# Autodesk Inventor assembly: PolarizationMethod
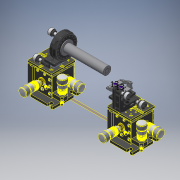
[picture p0: Inventor's stored thumbnail of the model, 180x180]
Saved by Autodesk Inventor 2019 (Build 230136000, 136)
## iProperties
Created: 2019-05-24
Part Number: PolarizationMethod
Document SubType Name: Assembly
Designer: aorfi
Author: aorfi
## Documents named in this file (10)
- C:\Users\aorfi\Documents\IQC\PolarizationMethod.iam
- C:\Users\aorfi\Documents\IQC\COTS\ThorLabs\3AxisStage-MBT616D.ipt
- C:\Users\aorfi\Documents\IQC\COTS\ThorLabs\RollStage-RSP1_M.ipt
- C:\Users\aorfi\Documents\IQC\COTS\ThorLabs\YawPitchStage-KM100PM.ipt
- C:\Users\aorfi\Documents\IQC\ChipMountAssembly.iam
- C:\Users\aorfi\Documents\IQC\COTS\Newport\LinearStage-MS-125-X.ipt
- C:\Users\aorfi\Documents\IQC\CustomParts\FiberMount.ipt
- C:\Users\aorfi\Documents\IQC\CustomParts\EpoxyFiberMountBase.ipt
- C:\Users\aorfi\Documents\IQC\CustomParts\FixedFiber.ipt
- C:\Users\aorfi\Documents\IQC\CustomParts\RubayetChip.ipt
## Components (12 placed, 9 different names)
1. 3AxisStage-MBT616D:1 — Mate:1, Flush:1, Mate:2, Flush:3, Flush:5
2. 3AxisStage-MBT616D:2 — Mate:6, Flush:4, Flush:5, Mate:8, Mate:12, Flush:7
3. RollStage-RSP1_M:1 — Mate:4, Angle:1, Mate:5, Mate:7, Mate:13, Mate:14
4. YawPitchStage-KM100PM:1 — Mate:2, Mate:4, Angle:1, Mate:13
5. ChipMountAssembly:1 [sub-assembly] — Mate:5, Mate:7
6. YawPitchStage-KM100PM:2 — Mate:8, Mate:10, Mate:12, Flush:6, Flush:7
7. LinearStage-MS-125-X:1 — Mate:10, Mate:11, Flush:6, Mate:16, Mate:17, Mate:18, Mate:19, Mate:20, Mate:21
8. FiberMount:1 — Mate:16, Flush:9, Mate:24, Mate:25, Mate:26, Flush:10
9. EpoxyFiberMountBase:1 — Mate:17, Mate:18, Mate:19, Flush:9, Mate:24
10. FixedFiber:1 — Mate:20, Mate:21, Mate:22, Mate:23, Flush:8
11. RubayetChip:1 — Mate:22, Mate:23, Flush:8
12. RubayetChip:2 — Mate:25, Mate:26, Flush:10
## Relationships (33: Mate 23, Flush 9, Angle 1)
- Mate:1: 3AxisStage-MBT616D:1
- Flush:1: 3AxisStage-MBT616D:1
- Mate:2: 3AxisStage-MBT616D:1 ↔ YawPitchStage-KM100PM:1
- Mate:4: RollStage-RSP1_M:1 ↔ YawPitchStage-KM100PM:1
- Flush:3: 3AxisStage-MBT616D:1
- Angle:1 (180 deg): RollStage-RSP1_M:1 ↔ YawPitchStage-KM100PM:1
- Mate:5: RollStage-RSP1_M:1 ↔ ChipMountAssembly:1
- Mate:6: 3AxisStage-MBT616D:2
- Flush:4: 3AxisStage-MBT616D:2
- Flush:5 (-200 mm): 3AxisStage-MBT616D:1 ↔ 3AxisStage-MBT616D:2
- Mate:7: RollStage-RSP1_M:1 ↔ ChipMountAssembly:1
- Mate:8: 3AxisStage-MBT616D:2 ↔ YawPitchStage-KM100PM:2
- Mate:10: YawPitchStage-KM100PM:2 ↔ LinearStage-MS-125-X:1
- Mate:11: LinearStage-MS-125-X:1
- Mate:12 (4 mm): 3AxisStage-MBT616D:2 ↔ YawPitchStage-KM100PM:2
- Flush:6: YawPitchStage-KM100PM:2 ↔ LinearStage-MS-125-X:1
- Flush:7: 3AxisStage-MBT616D:2 ↔ YawPitchStage-KM100PM:2
- Mate:13: RollStage-RSP1_M:1 ↔ YawPitchStage-KM100PM:1
- Mate:14: RollStage-RSP1_M:1
- Mate:16: LinearStage-MS-125-X:1 ↔ FiberMount:1
- Mate:17: LinearStage-MS-125-X:1 ↔ EpoxyFiberMountBase:1
- Mate:18: LinearStage-MS-125-X:1 ↔ EpoxyFiberMountBase:1
- Mate:19: LinearStage-MS-125-X:1 ↔ EpoxyFiberMountBase:1
- Mate:20: LinearStage-MS-125-X:1 ↔ FixedFiber:1
- Mate:21: LinearStage-MS-125-X:1 ↔ FixedFiber:1
- Mate:22: FixedFiber:1 ↔ RubayetChip:1
- Mate:23: FixedFiber:1 ↔ RubayetChip:1
- Flush:8: FixedFiber:1 ↔ RubayetChip:1
- Flush:9: FiberMount:1 ↔ EpoxyFiberMountBase:1
- Mate:24: FiberMount:1 ↔ EpoxyFiberMountBase:1
- Mate:25: FiberMount:1 ↔ RubayetChip:2
- Mate:26: FiberMount:1 ↔ RubayetChip:2
- Flush:10: FiberMount:1 ↔ RubayetChip:2
